# Autodesk Inventor assembly: 30 mm Eco Slider
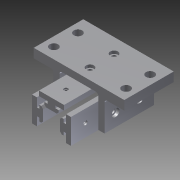
[picture p0: Inventor's stored thumbnail of the model, 180x180]
Saved by Autodesk Inventor 2013 (Build 170138000, 138)
## iProperties
Created: 2013-03-01
Part Number: 30 mm Eco Slider
Document SubType Name: Assembly
Designer: niemitalo_dan
Author: niemitalo_dan
## Documents named in this file (3)
- \\lmss\students\Robotics\CAD Files\COTS Parts\Bosch Extrusion\30 mm Eco Slider.iam
- \\lmss\students\Robotics\CAD Files\FRC 2013\Components\Eco Slider 30 mm cut down.ipt
- \\lmss\students\Robotics\CAD Files\FRC 2013\Components\30 mm plastic slider cut.ipt
## Components (4 placed, 2 different names)
1. Eco Slider 30 mm cut down:1 — Mate:4, Mate:5, Insert:1, Insert:2, Mate:6, Mate:7
2. 30 mm plastic slider cut:1 — Mate:4, Mate:5
3. 30 mm plastic slider cut:3 — Insert:1, Mate:6
4. 30 mm plastic slider cut:4 — Insert:2, Mate:7
## Relationships (7: Mate 5, Insert 2)
- [Mate]: Eco Slider 30 mm cut down:1 ↔ 30 mm plastic slider cut:1
- Mate:4: Eco Slider 30 mm cut down:1 ↔ 30 mm plastic slider cut:1
- Mate:5: Eco Slider 30 mm cut down:1 ↔ 30 mm plastic slider cut:1
- Insert:1: Eco Slider 30 mm cut down:1 ↔ 30 mm plastic slider cut:3
- Insert:2: Eco Slider 30 mm cut down:1 ↔ 30 mm plastic slider cut:4
- Mate:6: Eco Slider 30 mm cut down:1 ↔ 30 mm plastic slider cut:3
- Mate:7: Eco Slider 30 mm cut down:1 ↔ 30 mm plastic slider cut:4
